# Autodesk Inventor assembly: SC-4-F
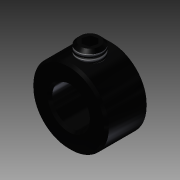
[picture p0: Inventor's stored thumbnail of the model, 180x180]
Saved by Autodesk Inventor 2014 (Build 180170000, 170)
## iProperties
Category: Miscellaneous
Company: Autodesk Inc.
Created: 2013-12-18
Part Number: SC-4-F
Document SubType Name: Assembly
Designer: Autodesk Inc.
Catalog Web Link: http://www.ruland.com/shaft-collar.php?recordID=SC-4-F
Vendor: Ruland Manufacturing
Description: 1/4" ID 1/2" OD Shaft collar
Author: Autodesk Inc.
## Documents named in this file (3)
- D:\Data Folder\FIRST 2014\KOP Parts\Miscellaneous\MISC_ShaftCollar_SC-4-F.iam
- D:\Data Folder\FIRST 2014\KOP Parts\Miscellaneous\MISC_ShaftCollar_SC-4-F.ipt
- D:\Data Folder\FIRST 2014\KOP Parts\Miscellaneous\ANSI B18.3 - 8-32 UNC - 0.19(24).ipt
## Components (2 placed, 2 different names)
1. MISC_ShaftCollar_SC-4-F:1 — Mate:1
2. Hexagon Socket Set Screw - Flat Point - Inch 8-32 UNC x 0.19:1 — Mate:1, Flush:1
## Relationships (2: Mate 1, Flush 1)
- Mate:1: MISC_ShaftCollar_SC-4-F:1 ↔ Hexagon Socket Set Screw - Flat Point - Inch 8-32 UNC x 0.19:1
- Flush:1 (-7.9375 mm): Hexagon Socket Set Screw - Flat Point - Inch 8-32 UNC x 0.19:1
